# Autodesk Inventor assembly: locomotion assembly
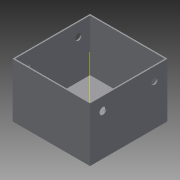
[picture p0: Inventor's stored thumbnail of the model, 180x180]
Saved by Autodesk Inventor 2015 (Build 190159000, 159)
## iProperties
Created: 2014-10-11
Part Number: locomotion assembly
Document SubType Name: Assembly
Designer: ericd_000
Author: ericd_000
## Documents named in this file (3)
- C:\Users\ericd_000\Dropbox\GitHub\initial_cad\eric_cad\locomotion assembly.iam
- C:\Users\ericd_000\Dropbox\GitHub\initial_cad\eric_cad\locomotion box.ipt
- C:\Users\ericd_000\Dropbox\GitHub\initial_cad\eric_cad\male bayonet connector 10.ipt
## Components (2 placed, 2 different names)
1. locomotion box:1 — Mate:1, Cylindrical:1, Cylindrical:2
2. male bayonet connector 10:1 — Mate:1, Cylindrical:1, Cylindrical:2
## Relationships (3: CylindricalJoint 2, Mate 1)
- Mate:1: locomotion box:1 ↔ male bayonet connector 10:1
- Cylindrical:1: locomotion box:1 ↔ male bayonet connector 10:1
- Cylindrical:2: locomotion box:1 ↔ male bayonet connector 10:1
